# Autodesk Inventor assembly: Mid Crossbrace
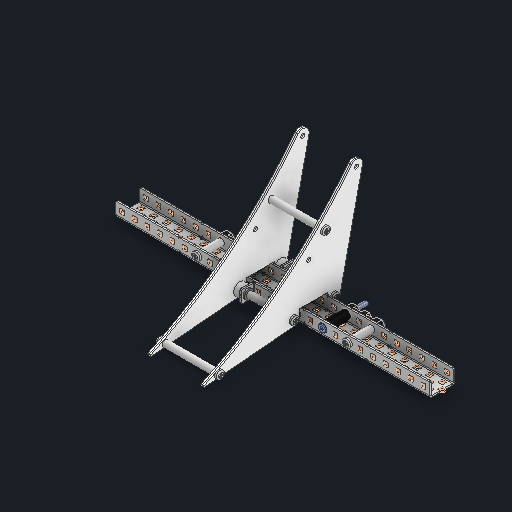
[picture p0: Inventor's stored thumbnail of the model, 512x512]
Saved by Autodesk Inventor 2025.1 (Build 291241000, 241)
## iProperties
Created: 2024-11-11
Part Number: Mid Crossbrace
Document SubType Name: Assembly
Designer: avere
Author: avere
## Documents named in this file (18)
- C:\Users\avere\VEX\High Stakes\CAD\V3\Chassis\Structure\Mid Crossbrace.iam
- C:\Users\avere\VEX\High Stakes\CAD\ROBOPROS-CAD-Inventor\Structure\C Channel\Aluminum 1x2x1\Alu C 1x2x1x25.ipt
- C:\Users\avere\VEX\High Stakes\CAD\ROBOPROS-CAD-Inventor\Structure\C Channel\Aluminum 1x3x1\Alu C 1x3x1x1.ipt
- C:\Users\avere\VEX\High Stakes\CAD\ROBOPROS-CAD-Inventor\Motion\Spacers\Spacer Nylon .500 OD\NSpacer White .500 OD x .250.ipt
- C:\Users\avere\VEX\High Stakes\CAD\ROBOPROS-CAD-Inventor\Motion\Spacers\Spacer Nylon .500 OD.ipt
- C:\Users\avere\VEX\High Stakes\CAD\V3\Chassis\Ramp\!Ramp.iam
- C:\Users\avere\VEX\High Stakes\CAD\ROBOPROS-CAD-Inventor\Structure\Hardware\Screw Nylon - Pan Head\NScrew Pan Head Threaded .750.ipt
- C:\Users\avere\VEX\High Stakes\CAD\ROBOPROS-CAD-Inventor\Motion\Spacers\Washer Steel\SWasher .375 OD x .062500.ipt
- C:\Users\avere\VEX\High Stakes\CAD\ROBOPROS-CAD-Inventor\Motion\Spacers\Washer Steel.ipt
- C:\Users\avere\VEX\High Stakes\CAD\ROBOPROS-CAD-Inventor\Structure\Nylon Standoff Rounded\Nylon Standoff 1.250.ipt
- C:\Users\avere\VEX\High Stakes\CAD\ROBOPROS-CAD-Inventor\Motion\Shaft LS\Bearing Flat.ipt
- C:\Users\avere\VEX\High Stakes\CAD\ROBOPROS-CAD-Inventor\Motion\Spacers\Spacer Nylon .375 OD\NSpacer .375 OD x .875.ipt
- C:\Users\avere\VEX\High Stakes\CAD\ROBOPROS-CAD-Inventor\Motion\Spacers\Spacer Nylon .375 OD.ipt
- C:\Users\avere\VEX\High Stakes\CAD\ROBOPROS-CAD-Inventor\Structure\Hardware\Screw Nylon - Pan Head\NScrew Pan Head Threaded .500.ipt
- C:\Users\avere\VEX\High Stakes\CAD\ROBOPROS-CAD-Inventor\Structure\Hardware\Screw Steel - Star.ipt
- C:\Users\avere\VEX\High Stakes\CAD\ROBOPROS-CAD-Inventor\Structure\Hardware\Screw Steel - Star\SScrew Star Smooth 1.750.ipt
- C:\Users\avere\VEX\High Stakes\CAD\ROBOPROS-CAD-Inventor\Structure\Hardware\Screw Nylon - Pan Head\NScrew Pan Head Threaded .250.ipt
- C:\Users\avere\VEX\High Stakes\CAD\ROBOPROS-CAD-Inventor\Structure\Nylon Standoff Rounded\Nylon Standoff .875.ipt
## Components (30 placed, 13 different names)
1. Alu C 1x2x1x25:1 — Mate:1, Mate:2, Mate:3, Insert:1, Mate:4, Insert:6, Mate:5, Insert:18, Mate:8, Insert:19, Insert:20, Mate:9, Insert:21, Insert:26, Insert:27, Insert:29, Insert:30, Insert:32, Insert:33
2. Alu C 1x3x1x1:1 — Insert:1, Mate:4, Insert:2, Insert:3, Insert:16
3. NSpacer White .500 OD x .250:1 — Insert:3, Insert:7
4. NSpacer White .500 OD x .250:2 — Insert:2, Mate:6
5. Alu C 1x3x1x1:2 — Insert:6, Mate:5, Insert:12, Insert:13
6. NSpacer White .500 OD x .250:3
7. NSpacer White .500 OD x .250:4 — Mate:7
8. !Ramp:1 [sub-assembly] — Insert:7, Mate:6, Mate:7, Insert:8, Insert:9, Insert:10, Insert:11
9. NScrew Pan Head Threaded .750:1 — Insert:8
10. NScrew Pan Head Threaded .750:2 — Insert:9
11. NScrew Pan Head Threaded .750:3 — Insert:10
12. NScrew Pan Head Threaded .750:4 — Insert:11
13. SWasher .375 OD x .062500:1 — Insert:12
14. SWasher .375 OD x .062500:2 — Insert:13, Insert:14
15. Nylon Standoff 1.250:1 — Insert:14
16. SWasher .375 OD x .062500:4 — Insert:16
17. Nylon Standoff 1.250:2 — Insert:17
18. SWasher .375 OD x .062500:5 — Insert:17
19. Bearing Flat:1 — Insert:18, Mate:8, Insert:28
20. NSpacer .375 OD x .875:1 — Insert:19
21. Bearing Flat:2 — Insert:20, Mate:9, Insert:31
22. NSpacer .375 OD x .875:2 — Insert:21
23. NScrew Pan Head Threaded .500:1 — Insert:28
24. SScrew Star Smooth 1.750:1 — Insert:26
25. SScrew Star Smooth 1.750:2 — Insert:27
26. NScrew Pan Head Threaded .250:1 — Insert:29
27. Nylon Standoff .875:1 — Insert:30
28. NScrew Pan Head Threaded .500:3 — Insert:31
29. NScrew Pan Head Threaded .250:2 — Insert:33
30. Nylon Standoff .875:2 — Insert:32
## Relationships (38: Insert 29, Mate 9)
- Mate:1 (-158.75 mm): Alu C 1x2x1x25:1
- Mate:2 (7.9375 mm): Alu C 1x2x1x25:1
- Mate:3 (63.4238 mm): Alu C 1x2x1x25:1
- Insert:1: Alu C 1x2x1x25:1 ↔ Alu C 1x3x1x1:1
- Mate:4: Alu C 1x2x1x25:1 ↔ Alu C 1x3x1x1:1
- Insert:2: Alu C 1x3x1x1:1 ↔ NSpacer White .500 OD x .250:2
- Insert:3: Alu C 1x3x1x1:1 ↔ NSpacer White .500 OD x .250:1
- [Insert]: Alu C 1x3x1x1:2 ↔ NSpacer White .500 OD x .250:4
- [Insert]: Alu C 1x3x1x1:2 ↔ NSpacer White .500 OD x .250:3
- Insert:6: Alu C 1x2x1x25:1 ↔ Alu C 1x3x1x1:2
- Mate:5: Alu C 1x2x1x25:1 ↔ Alu C 1x3x1x1:2
- Insert:7: NSpacer White .500 OD x .250:1 ↔ !Ramp:1
- Mate:6: NSpacer White .500 OD x .250:2 ↔ !Ramp:1
- Mate:7: NSpacer White .500 OD x .250:4 ↔ !Ramp:1
- Insert:8: !Ramp:1 ↔ NScrew Pan Head Threaded .750:1
- Insert:9: !Ramp:1 ↔ NScrew Pan Head Threaded .750:2
- Insert:10: !Ramp:1 ↔ NScrew Pan Head Threaded .750:3
- Insert:11: !Ramp:1 ↔ NScrew Pan Head Threaded .750:4
- Insert:12: Alu C 1x3x1x1:2 ↔ SWasher .375 OD x .062500:1
- Insert:13: Alu C 1x3x1x1:2 ↔ SWasher .375 OD x .062500:2
- Insert:14: SWasher .375 OD x .062500:2 ↔ Nylon Standoff 1.250:1
- [Insert]: SWasher .375 OD x .062500:4 ↔ Nylon Standoff 1.250:2
- Insert:16: Alu C 1x3x1x1:1 ↔ SWasher .375 OD x .062500:4
- Insert:17: Nylon Standoff 1.250:2 ↔ SWasher .375 OD x .062500:5
- Insert:18: Alu C 1x2x1x25:1 ↔ Bearing Flat:1
- Mate:8: Alu C 1x2x1x25:1 ↔ Bearing Flat:1
- Insert:19: Alu C 1x2x1x25:1 ↔ NSpacer .375 OD x .875:1
- Insert:20: Alu C 1x2x1x25:1 ↔ Bearing Flat:2
- Mate:9: Alu C 1x2x1x25:1 ↔ Bearing Flat:2
- Insert:21: Alu C 1x2x1x25:1 ↔ NSpacer .375 OD x .875:2
- Insert:26: Alu C 1x2x1x25:1 ↔ SScrew Star Smooth 1.750:1
- Insert:27: Alu C 1x2x1x25:1 ↔ SScrew Star Smooth 1.750:2
- Insert:28: Bearing Flat:1 ↔ NScrew Pan Head Threaded .500:1
- Insert:29: Alu C 1x2x1x25:1 ↔ NScrew Pan Head Threaded .250:1
- Insert:30: Alu C 1x2x1x25:1 ↔ Nylon Standoff .875:1
- Insert:31: Bearing Flat:2 ↔ NScrew Pan Head Threaded .500:3
- Insert:32: Alu C 1x2x1x25:1 ↔ Nylon Standoff .875:2
- Insert:33: Alu C 1x2x1x25:1 ↔ NScrew Pan Head Threaded .250:2
## Named parameters: d7_d5 = 0 mm, d8_d6 = 0 mm, d32_d31 = 0 mm
